# Autodesk Inventor assembly: Assembly_Matchboxscope_injectionmolded_motorized
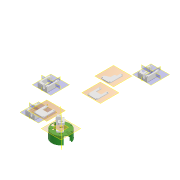
[picture p0: Inventor's stored thumbnail of the model, 180x180]
Saved by Autodesk Inventor 2022 (Build 260153000, 153)
## iProperties
Created: 2023-08-15
Part Number: Assembly_Matchboxscope_injectionmolded_motorized
Document SubType Name: Assembly
Designer: diederichbenedict
Author: diederichbenedict
## Documents named in this file (9)
- C:\Users\diederichbenedict\Dropbox\Dokumente\Promotion\PROJECTS\Matchboxscope\INVENTOR\RELEASE\InjectionMolded\Assembly_Matchboxscope_injectionmolded_motorized.iam
- C:\Users\diederichbenedict\Dropbox\Dokumente\Promotion\PROJECTS\Matchboxscope\INVENTOR\RELEASE\InjectionMolded\IM_Matchboxscope_base_old.ipt
- C:\Users\diederichbenedict\Dropbox\Dokumente\Promotion\PROJECTS\Matchboxscope\INVENTOR\RELEASE\InjectionMolded\00_Microlinearmotor.ipt
- C:\Users\diederichbenedict\Dropbox\Dokumente\Promotion\PROJECTS\Matchboxscope\INVENTOR\RELEASE\InjectionMolded\IM_Lensholder_motorized.ipt
- C:\Users\diederichbenedict\Dropbox\Dokumente\Promotion\PROJECTS\Matchboxscope\INVENTOR\RELEASE\InjectionMolded\IM_Lensholder_motorized_lensadapter.ipt
- C:\Users\diederichbenedict\Dropbox\Dokumente\Promotion\PROJECTS\Matchboxscope\INVENTOR\RELEASE\InjectionMolded\00_ESP32_XIAO_Adapter_base.ipt
- C:\Users\diederichbenedict\Dropbox\Dokumente\Promotion\PROJECTS\Matchboxscope\INVENTOR\RELEASE\InjectionMolded\00_ESP32_XIAO_Adapter_lid.ipt
- C:\Users\diederichbenedict\Dropbox\Dokumente\Promotion\PROJECTS\Matchboxscope\INVENTOR\RELEASE\InjectionMolded\00_ESP32_XIAO_Adapter_base_a4988.ipt
- C:\Users\diederichbenedict\Dropbox\Dokumente\Promotion\PROJECTS\Matchboxscope\INVENTOR\RELEASE\InjectionMolded\00_ESP32_XIAO_Adapter_lid_a4988.ipt
## Components (10 placed, 8 different names)
1. IM_Matchboxscope_base_old:1 — Einfügen:1, Winkel:1, Fluchtend:1
2. 00_Microlinearmotor:1 — Einfügen:1, Winkel:1, Fluchtend:2
3. IM_Lensholder_motorized:1 — Fluchtend:1
4. IM_Lensholder_motorized_lensadapter:1 — Fluchtend:2
5. 00_ESP32_XIAO_Adapter_lid:1
6. 00_ESP32_XIAO_Adapter_base:1
7. 00_ESP32_XIAO_Adapter_lid:2
8. 00_ESP32_XIAO_Adapter_base_a4988:1
9. 00_ESP32_XIAO_Adapter_lid_a4988:1
10. 00_ESP32_XIAO_Adapter_base_a4988:2
## Relationships (4: Flush 2, Insert 1, Angle 1)
- Einfügen:1 [Insert]: IM_Matchboxscope_base_old:1 ↔ 00_Microlinearmotor:1
- Winkel:1 [Angle] (90 deg): IM_Matchboxscope_base_old:1 ↔ 00_Microlinearmotor:1
- Fluchtend:1 [Flush]: IM_Matchboxscope_base_old:1 ↔ IM_Lensholder_motorized:1
- Fluchtend:2 [Flush]: 00_Microlinearmotor:1 ↔ IM_Lensholder_motorized_lensadapter:1
